# Autodesk Inventor assembly: X-axis assy
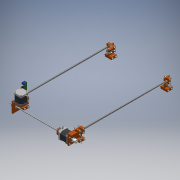
[picture p0: Inventor's stored thumbnail of the model, 180x180]
Saved by Autodesk Inventor 2018 (Build 220112000, 112)
## iProperties
Created: 2017-10-27
Part Number: X-axis assy
Document SubType Name: Assembly
Designer: Gabriel Smolnycki
Author: Gabriel Smolnycki
## Documents named in this file (14)
- H:\dev\planb\mechanics\V1INV\Subassemblies\X-axis assy.iam
- H:\dev\planb\mechanics\V1INV\Subassemblies\X-axis Idler 1 assy.iam
- H:\dev\planb\mechanics\V1INV\X-axis\X-axis Rod 8mm.ipt
- H:\dev\planb\mechanics\V1INV\Subassemblies\X-axis Motor Holder assy.iam
- H:\dev\planb\mechanics\V1INV\X-axis\X-axis Axle 5mm.ipt
- H:\dev\planb\mechanics\V1INV\X-axis\X-axis Driver Clamp.ipt
- H:\dev\planb\mechanics\V1INV\Hardware\M4 SS Washer.ipt
- H:\dev\planb\mechanics\V1INV\Hardware\M4 SS Locknut.ipt
- H:\dev\planb\mechanics\V1INV\Hardware\M4x20 SS SHCS.ipt
- H:\dev\planb\mechanics\V1INV\Hardware\M4x25 SS SHCS.ipt
- H:\dev\planb\mechanics\V1INV\Subassemblies\X-axis Y-axis Motor Holder assy.iam
- H:\dev\planb\mechanics\V1INV\Subassemblies\X-axis Driver Holder assy.iam
- H:\dev\planb\mechanics\V1INV\Hardware\T2.5 16T Pulley.ipt
- H:\dev\planb\mechanics\V1INV\Subassemblies\X-axis Idler 2 assy.iam
## Components (35 placed, 13 different names)
1. X-axis Idler 1 assy:1 [sub-assembly] — Insert:1, Flush:1
2. X-axis Rod 8mm:1 — Insert:1, Insert:2
3. X-axis Motor Holder assy:1 [sub-assembly] — Insert:2, Flush:1, Insert:3, Flush:2, Insert:5, Flush:4
4. X-axis Axle 5mm:1 — Insert:5, Insert:22
5. X-axis Driver Clamp:1 — Insert:3, Flush:2, Flush:3, Insert:4, Mate:1, Insert:14, Insert:15, Insert:16, Insert:17
6. X-axis Driver Clamp:2 — Flush:3, Insert:4, Mate:1, Insert:18, Insert:19, Insert:20, Insert:21
7. M4 SS Washer:1 — Insert:14
8. M4 SS Washer:2 — Insert:7, Insert:18
9. M4 SS Locknut:1 — Insert:7
10. M4x25 SS SHCS:4
11. M4 SS Washer:3 — Insert:15
12. M4 SS Washer:4 — Insert:20
13. M4 SS Locknut:2
14. M4x25 SS SHCS:3
15. M4 SS Washer:5 — Insert:16
16. M4 SS Washer:6 — Insert:21
17. M4 SS Locknut:3
18. M4x25 SS SHCS:2
19. M4 SS Washer:7 — Insert:17
20. M4 SS Washer:8 — Insert:19
21. M4 SS Locknut:4
22. M4x25 SS SHCS:1
23. X-axis Y-axis Motor Holder assy:1 [sub-assembly] — Insert:24, Insert:25, Insert:28, Insert:29
24. X-axis Driver Holder assy:1 [sub-assembly] — Insert:23, Insert:24, Insert:25, Flush:4, Insert:32, Insert:33, Insert:34
25. T2.5 16T Pulley:1 — Insert:22, Insert:23
26. M4 SS Washer:9 — Insert:28
27. M4x20 SS SHCS:2
28. M4 SS Washer:10 — Insert:29
29. M4x20 SS SHCS:1
30. M4 SS Washer:11 — Insert:32
31. M4 SS Locknut:5
32. M4 SS Washer:12 — Insert:33
33. M4 SS Locknut:6
34. X-axis Rod 8mm:2 — Insert:34, Insert:35
35. X-axis Idler 2 assy:1 [sub-assembly] — Insert:35
## Relationships (40: Insert 35, Flush 4, Mate 1)
- Insert:1 (-8 mm): X-axis Idler 1 assy:1 ↔ X-axis Rod 8mm:1
- Insert:2: X-axis Rod 8mm:1 ↔ X-axis Motor Holder assy:1
- Flush:1: X-axis Idler 1 assy:1 ↔ X-axis Motor Holder assy:1
- Insert:3 (10 mm): X-axis Motor Holder assy:1 ↔ X-axis Driver Clamp:1
- Flush:2: X-axis Motor Holder assy:1 ↔ X-axis Driver Clamp:1
- Flush:3: X-axis Driver Clamp:1 ↔ X-axis Driver Clamp:2
- Insert:4: X-axis Driver Clamp:1 ↔ X-axis Driver Clamp:2
- Mate:1: X-axis Driver Clamp:1 ↔ X-axis Driver Clamp:2
- Insert:5: X-axis Motor Holder assy:1 ↔ X-axis Axle 5mm:1
- [Insert]: M4 SS Washer:1 ↔ M4x25 SS SHCS:4
- Insert:7: M4 SS Washer:2 ↔ M4 SS Locknut:1
- [Insert]: M4 SS Washer:3 ↔ M4x25 SS SHCS:3
- [Insert]: M4 SS Washer:4 ↔ M4 SS Locknut:2
- [Insert]: M4 SS Washer:5 ↔ M4x25 SS SHCS:2
- [Insert]: M4 SS Washer:6 ↔ M4 SS Locknut:3
- [Insert]: M4 SS Washer:7 ↔ M4x25 SS SHCS:1
- [Insert]: M4 SS Washer:8 ↔ M4 SS Locknut:4
- Insert:14: X-axis Driver Clamp:1 ↔ M4 SS Washer:1
- Insert:15: X-axis Driver Clamp:1 ↔ M4 SS Washer:3
- Insert:16: X-axis Driver Clamp:1 ↔ M4 SS Washer:5
- Insert:17: X-axis Driver Clamp:1 ↔ M4 SS Washer:7
- Insert:18: X-axis Driver Clamp:2 ↔ M4 SS Washer:2
- Insert:19: X-axis Driver Clamp:2 ↔ M4 SS Washer:8
- Insert:20: X-axis Driver Clamp:2 ↔ M4 SS Washer:4
- Insert:21: X-axis Driver Clamp:2 ↔ M4 SS Washer:6
- Insert:22 (-13.5 mm): X-axis Axle 5mm:1 ↔ T2.5 16T Pulley:1
- Insert:23: X-axis Driver Holder assy:1 ↔ T2.5 16T Pulley:1
- Insert:24: X-axis Y-axis Motor Holder assy:1 ↔ X-axis Driver Holder assy:1
- Insert:25: X-axis Y-axis Motor Holder assy:1 ↔ X-axis Driver Holder assy:1
- Flush:4: X-axis Motor Holder assy:1 ↔ X-axis Driver Holder assy:1
- [Insert]: M4 SS Washer:9 ↔ M4x20 SS SHCS:2
- [Insert]: M4 SS Washer:10 ↔ M4x20 SS SHCS:1
- Insert:28: X-axis Y-axis Motor Holder assy:1 ↔ M4 SS Washer:9
- Insert:29: X-axis Y-axis Motor Holder assy:1 ↔ M4 SS Washer:10
- [Insert]: M4 SS Washer:11 ↔ M4 SS Locknut:5
- [Insert]: M4 SS Washer:12 ↔ M4 SS Locknut:6
- Insert:32: X-axis Driver Holder assy:1 ↔ M4 SS Washer:11
- Insert:33: X-axis Driver Holder assy:1 ↔ M4 SS Washer:12
- Insert:34: X-axis Driver Holder assy:1 ↔ X-axis Rod 8mm:2
- Insert:35 (8 mm): X-axis Rod 8mm:2 ↔ X-axis Idler 2 assy:1
## Named parameters: d19_d17 = 0 mm, d20_d18 = 0 mm, d21_d17 = 0 mm, d22_d18 = 0 mm, d23_d17 = 0 mm, d24_d18 = 0 mm, d38_d23_d17 = 0 mm, d39_d38_d23_d17 = 0 mm, d42_d24_d18 = 0 mm, d43_d24_d18 = 0 mm
